# Autodesk Inventor assembly: Button2
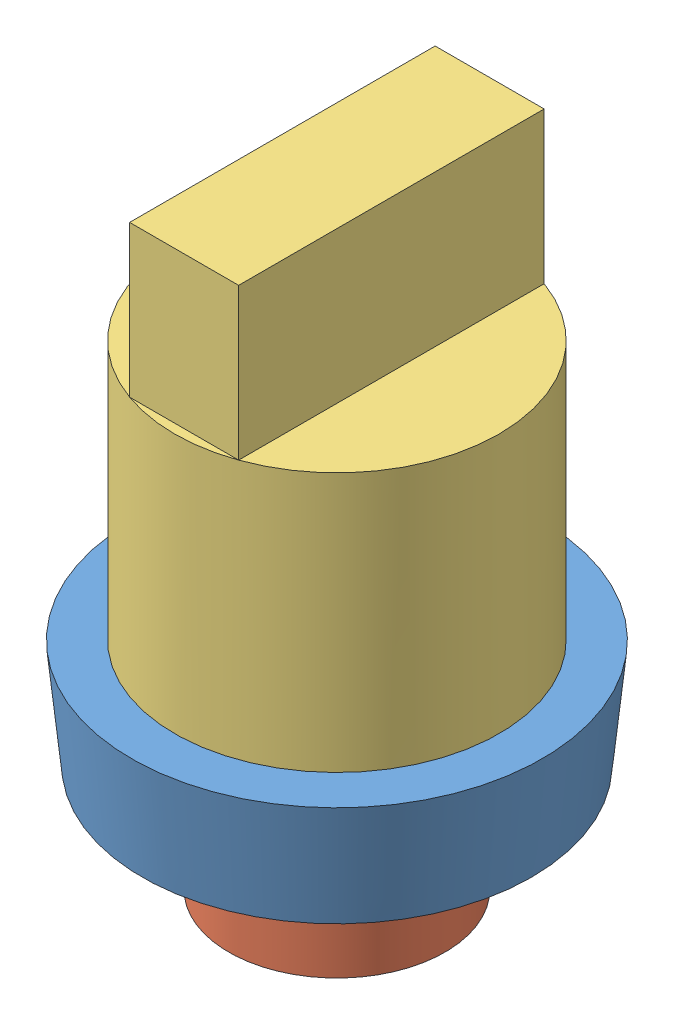
[picture p0: shaded view drawn from the part files that the assembly names]
Saved by Autodesk Inventor 2015 (Build 190159000, 159)
## iProperties
Created: 2016-01-04
Part Number: Button2
Document SubType Name: Assembly
Designer: david
Author: david
## Documents named in this file (4)
- Z:\gip\Inventor\generatie 7\Frame\doos\Button2.iam
- Z:\gip\Inventor\generatie 7\Frame\doos\kop.ipt
- Z:\gip\Inventor\generatie 7\Frame\doos\Button.ipt
- Z:\gip\Inventor\generatie 7\Frame\doos\voet.ipt
## Components (3 placed, 3 different names)
1. kop:1 — Mate:1, Mate:2, Mate:3, Mate:4
2. Button:1 — Mate:1, Mate:2
3. voet:1 — Mate:3, Mate:4
## Relationships (4: Mate 4)
- Mate:1: kop:1 ↔ Button:1
- Mate:2 (-1 mm): kop:1 ↔ Button:1
- Mate:3: kop:1 ↔ voet:1
- Mate:4: kop:1 ↔ voet:1
